# Autodesk Inventor assembly: Cartridge PCB Assembly
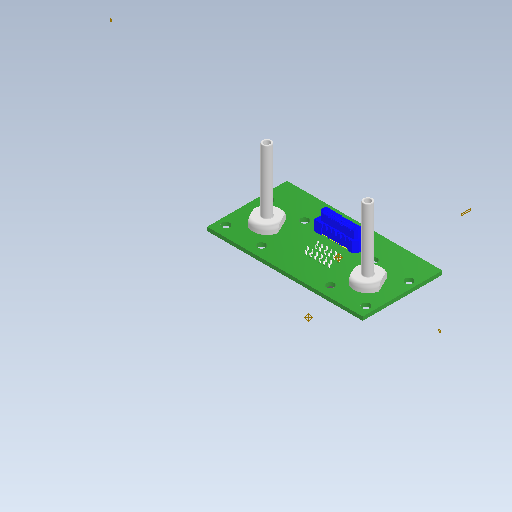
[picture p0: Inventor's stored thumbnail of the model, 512x512]
Saved by Autodesk Inventor 2021 (Build 250183000, 183)
## iProperties
Created: 2020-04-23
Part Number: Cartridge PCB Assembly
Document SubType Name: Assembly
Designer: jgray
Author: jgray
## Documents named in this file (7)
- M:\Printed Electronics\Gas Sensors\Prototypes\Prototype II -Cartridge Reader V2\Cartridge Interface V5 30-06-20\Cartridge PCB Assembly.iam
- M:\Printed Electronics\Gas Sensors\Prototypes\Prototype II -Cartridge Reader V2\Cartridge Interface V5 30-06-20\Digikey H125539CT-NDER8-30P-0.8SV-5H_TOP.iam
- M:\Printed Electronics\Gas Sensors\Prototypes\Prototype II -Cartridge Reader V2\Cartridge Interface V5 30-06-20\Cartridge PCB.ipt
- M:\Printed Electronics\Gas Sensors\Prototypes\Prototype II -Cartridge Reader V2\Cartridge Interface V5 30-06-20\DigiKey609-1939-ND islw12s-1c7_lf.ipt
- M:\Printed Electronics\Gas Sensors\Prototypes\Prototype II -Cartridge Reader V2\Cartridge Interface V5 30-06-20\Cartridge Tube Seal.iam
- M:\Printed Electronics\Gas Sensors\Prototypes\Prototype II -Cartridge Reader V2\Cartridge Interface V5 30-06-20\RS 122-4022 StSt304 Half Nut DIN 439 - M5 x 0.8.ipt
- M:\Printed Electronics\Gas Sensors\Prototypes\Prototype II -Cartridge Reader V2\Cartridge Interface V5 30-06-20\RS 665-7302  DIN 6798 - J  M5 tooth washer 0-6 Thk.ipt
## Components (10 placed, 6 different names)
1. Digikey H125539CT-NDER8-30P-0.8SV-5H_TOP:1 [sub-assembly] — Mate:1, Mate:2, Angle:1
2. Cartridge PCB:1 — Mate:1, Mate:2, Angle:1, Mate:9, Flush:5, Angle:2, Flush:6, Mate:10, Angle:3, Mate:17, Mate:18, Mate:19, Mate:20, Mate:21, Mate:22, Angle:24, Angle:25
3. DigiKey609-1939-ND islw12s-1c7_lf:1 — Flush:3, Flush:4, Flush:5, Angle:2
4. DigiKey609-1939-ND islw12s-1c7_lf:2 — Flush:1, Flush:2, Mate:3, Flush:6, Angle:3
5. Cartridge Tube Seal:1 [sub-assembly] — Mate:18, Mate:19
6. DIN 439-2 - replaced by DIN EN 24035/28675 M5:1
7. DIN 6798 J J 5.3:1 — Mate:20
8. Cartridge Tube Seal:2 [sub-assembly] — Mate:17, Mate:21
9. DIN 439-2 - replaced by DIN EN 24035/28675 M5:2
10. DIN 6798 J J 5.3:2 — Mate:22
## Relationships (32: Mate 21, Flush 6, Angle 5)
- Mate:1 (0.01 mm): Digikey H125539CT-NDER8-30P-0.8SV-5H_TOP:1 ↔ Cartridge PCB:1
- Mate:2: Digikey H125539CT-NDER8-30P-0.8SV-5H_TOP:1 ↔ Cartridge PCB:1
- Angle:1 (0 deg): Digikey H125539CT-NDER8-30P-0.8SV-5H_TOP:1 ↔ Cartridge PCB:1
- Flush:1 (0.125 mm): DigiKey609-1939-ND islw12s-1c7_lf:2
- Flush:2 (-0.25 mm): DigiKey609-1939-ND islw12s-1c7_lf:2
- Mate:3: DigiKey609-1939-ND islw12s-1c7_lf:2
- Mate:4
- Mate:5
- Flush:3 (-0.25 mm): DigiKey609-1939-ND islw12s-1c7_lf:1
- Flush:4 (0.125 mm): DigiKey609-1939-ND islw12s-1c7_lf:1
- Mate:6
- Mate:8
- Mate:9: Cartridge PCB:1
- Flush:5: Cartridge PCB:1 ↔ DigiKey609-1939-ND islw12s-1c7_lf:1
- Angle:2 (180 deg): Cartridge PCB:1 ↔ DigiKey609-1939-ND islw12s-1c7_lf:1
- Flush:6: Cartridge PCB:1 ↔ DigiKey609-1939-ND islw12s-1c7_lf:2
- Mate:10: Cartridge PCB:1
- Angle:3 (0 deg): Cartridge PCB:1 ↔ DigiKey609-1939-ND islw12s-1c7_lf:2
- [Mate]: Cartridge Tube Seal:1 ↔ DIN 6798 J J 5.3:1
- [Mate]: DIN 439-2 - replaced by DIN EN 24035/28675 M5:1 ↔ DIN 6798 J J 5.3:1
- [Mate]: Cartridge Tube Seal:1 ↔ DIN 439-2 - replaced by DIN EN 24035/28675 M5:1
- [Mate]: Cartridge Tube Seal:2 ↔ DIN 6798 J J 5.3:2
- [Mate]: DIN 439-2 - replaced by DIN EN 24035/28675 M5:2 ↔ DIN 6798 J J 5.3:2
- [Mate]: Cartridge Tube Seal:2 ↔ DIN 439-2 - replaced by DIN EN 24035/28675 M5:2
- Mate:17: Cartridge PCB:1 ↔ Cartridge Tube Seal:2
- Mate:18: Cartridge PCB:1 ↔ Cartridge Tube Seal:1
- Mate:19: Cartridge PCB:1 ↔ Cartridge Tube Seal:1
- Mate:20: Cartridge PCB:1 ↔ DIN 6798 J J 5.3:1
- Mate:21: Cartridge PCB:1 ↔ Cartridge Tube Seal:2
- Mate:22: Cartridge PCB:1 ↔ DIN 6798 J J 5.3:2
- Angle:24 (0 deg): Cartridge PCB:1
- Angle:25 (0 deg): Cartridge PCB:1
## Named parameters: d22_d17 = 0 mm, d23_d18 = 0 mm, d24_d13 = 0 mm, d25_d17 = 0 mm, d26_d18 = 0 mm
